# Autodesk Inventor assembly: 2020corner-assmbly_MIR2_MIR_MIR2
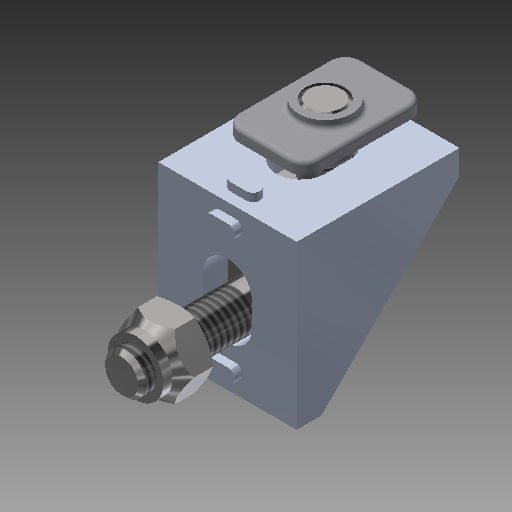
[picture p0: Inventor's stored thumbnail of the model, 512x512]
Saved by Autodesk Inventor 2017 (Build 210142000, 142)
## iProperties
Created: 2016-07-20
Part Number: 2020corner-assmbly_MIR2_MIR_MIR2
Document SubType Name: Assembly
Designer: User
Author: User
## Documents named in this file (6)
- C:\All INVENTOR\SL-Inventor\SL-Beast 3D Printer\2020corner-assmbly_MIR2_MIR_MIR2.iam
- C:\All INVENTOR\SL-Inventor\SL-Beast 3D Printer\20mm Bracket_MIR1_MIR_MIR2.ipt
- C:\All INVENTOR\SL-Inventor\SL-Beast 3D Printer\en-US\ANSI B18.3.1M(6)\ANSI B18.3.1M - M5x0.8 x 8(1).ipt
- C:\All INVENTOR\SL-Inventor\SL-Beast 3D Printer\M5 Tee Nut_MIR_MIR_MIR5.ipt
- C:\All INVENTOR\SL-Inventor\SL-Beast 3D Printer\en-US\ANSI B18.3.1M(6)\ANSI B18.3.1M - M5x0.8 x 16(1).ipt
- C:\All INVENTOR\SL-Inventor\SL-Beast 3D Printer\en-US\ANSI B18.16.3M(2)\ANSI B18.16.3M - Property Class 9 - Metric M5 x 0.8 Metal Type.ipt
## Components (5 placed, 5 different names)
1. 20mm Bracket_MIR1_MIR_MIR2:1 — Insert:1, Mate:2, Angle:1, Insert:2, Mate:4
2. Forged Socket Head Cap Screw - Metric M5x0.8 x 8:1 — Insert:1, Mate:1
3. M5 Tee Nut_MIR_MIR_MIR5:1 — Mate:2, Angle:1, Mate:1
4. Forged Socket Head Cap Screw - Metric M5x0.8 x 16:1 — Insert:2, Mate:3
5. Prevailing Torque Type Hex Nut - Steel Metric Property Class 9 - Metric M5 x 0.8 Metal Type:1 — Mate:4, Mate:3
## Relationships (7: Mate 4, Insert 2, Angle 1)
- Insert:1: 20mm Bracket_MIR1_MIR_MIR2:1 ↔ Forged Socket Head Cap Screw - Metric M5x0.8 x 8:1
- Mate:2 (2.5 mm): 20mm Bracket_MIR1_MIR_MIR2:1 ↔ M5 Tee Nut_MIR_MIR_MIR5:1
- Angle:1 (0 deg): 20mm Bracket_MIR1_MIR_MIR2:1 ↔ M5 Tee Nut_MIR_MIR_MIR5:1
- Mate:1: Forged Socket Head Cap Screw - Metric M5x0.8 x 8:1 ↔ M5 Tee Nut_MIR_MIR_MIR5:1
- Insert:2: 20mm Bracket_MIR1_MIR_MIR2:1 ↔ Forged Socket Head Cap Screw - Metric M5x0.8 x 16:1
- Mate:4 (6 mm): 20mm Bracket_MIR1_MIR_MIR2:1 ↔ Prevailing Torque Type Hex Nut - Steel Metric Property Class 9 - Metric M5 x 0.8 Metal Type:1
- Mate:3: Forged Socket Head Cap Screw - Metric M5x0.8 x 16:1 ↔ Prevailing Torque Type Hex Nut - Steel Metric Property Class 9 - Metric M5 x 0.8 Metal Type:1
